# Autodesk Inventor assembly: serre
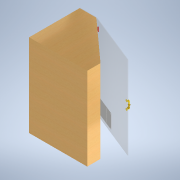
[picture p0: Inventor's stored thumbnail of the model, 180x180]
Saved by Autodesk Inventor 2022 (Build 260153000, 153)
## iProperties
Created: 2022-08-02
Part Number: serre
Document SubType Name: Assembly
Designer: thoma
Author: thoma
## Documents named in this file (7)
- C:\Users\thoma\OneDrive\Documents\CREATION\Serre\serre.iam
- C:\Users\thoma\OneDrive\Documents\CREATION\Serre\bois.ipt
- C:\Users\thoma\OneDrive\Documents\CREATION\Serre\plafond.ipt
- C:\Users\thoma\OneDrive\Documents\CREATION\Serre\capot.ipt
- C:\Users\thoma\OneDrive\Documents\CREATION\Serre\poigne.ipt
- C:\Users\thoma\OneDrive\Documents\CREATION\Serre\halfhinge.ipt
- C:\Users\thoma\OneDrive\Documents\CREATION\Serre\solar_panel.ipt
## Components (9 placed, 6 different names)
1. bois:1 — Flush:1, Flush:4, Flush:5
2. plafond:1 — Flush:1, Flush:4, Flush:5, Flush:7, Mate:2, Flush:8, Mate:6, Flush:11, Flush:12
3. capot:1 — Mate:1, Angle:1, Flush:3, Flush:6, Flush:9, Mate:3, Flush:10, Mate:7, Flush:13, Flush:14, Mate:8, Mate:9, Mate:10
4. poigne:1 — Mate:1, Angle:1, Flush:3, Flush:6
5. halfhinge:1 — Flush:7, Mate:2, Flush:8, Mate:4, Mate:5
6. halfhinge:2 — Flush:9, Mate:3, Flush:10, Mate:4, Mate:5
7. halfhinge:3 — Mate:6, Flush:11, Flush:12
8. halfhinge:4 — Mate:7, Flush:13, Flush:14
9. solar_panel:1 — Mate:8, Mate:9, Mate:10
## Relationships (24: Flush 13, Mate 10, Angle 1)
- Flush:1: bois:1 ↔ plafond:1
- Mate:1: capot:1 ↔ poigne:1
- Angle:1 (0 deg): capot:1 ↔ poigne:1
- Flush:3 (40 mm): capot:1 ↔ poigne:1
- Flush:4: bois:1 ↔ plafond:1
- Flush:5: bois:1 ↔ plafond:1
- Flush:6 (-450 mm): capot:1 ↔ poigne:1
- Flush:7 (100 mm): plafond:1 ↔ halfhinge:1
- Mate:2: plafond:1 ↔ halfhinge:1
- Flush:8: plafond:1 ↔ halfhinge:1
- Flush:9: capot:1 ↔ halfhinge:2
- Mate:3: capot:1 ↔ halfhinge:2
- Flush:10 (100 mm): capot:1 ↔ halfhinge:2
- Mate:4 (0.6 mm): halfhinge:1 ↔ halfhinge:2
- Mate:5: halfhinge:1 ↔ halfhinge:2
- Mate:6: plafond:1 ↔ halfhinge:3
- Flush:11 (100 mm): plafond:1 ↔ halfhinge:3
- Flush:12: plafond:1 ↔ halfhinge:3
- Mate:7: capot:1 ↔ halfhinge:4
- Flush:13 (100 mm): capot:1 ↔ halfhinge:4
- Flush:14: capot:1 ↔ halfhinge:4
- Mate:8: capot:1 ↔ solar_panel:1
- Mate:9 (-10 mm): capot:1 ↔ solar_panel:1
- Mate:10 (-10 mm): capot:1 ↔ solar_panel:1
